# Autodesk Inventor assembly: Tamale Assembly Plate Assembly V3
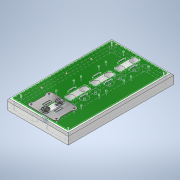
[picture p0: Inventor's stored thumbnail of the model, 180x180]
Saved by Autodesk Inventor 2022 (Build 260153000, 153)
## iProperties
Created: 2022-03-23
Part Number: Tamale Assembly Plate Assembly V3
Document SubType Name: Assembly
Designer: Caleb
Author: Caleb
## Documents named in this file (7)
- C:\Users\Caleb\Desktop\nebraska-silicon-lab\Hardware\ETL\Module Assembly\Tamale Assembly Plate V3\Tamale Assembly Plate Assembly V3.iam
- C:\Users\Caleb\Desktop\nebraska-silicon-lab\Hardware\ETL\Module Assembly\Tamale Assembly Plate V3\Tamale Assembly Plate V3.ipt
- C:\Users\Caleb\Desktop\nebraska-silicon-lab\Hardware\ETL\Module Assembly\Tamale Assembly Plate V3\5427A624_Vacuum Cup.ipt
- C:\Users\Caleb\Desktop\nebraska-silicon-lab\Hardware\ETL\Module Assembly\Tamale Assembly Plate V3\spacer.ipt
- C:\Users\Caleb\Desktop\nebraska-silicon-lab\Hardware\ETL\Module Assembly\Tamale Assembly Plate V3\Assembly Plate PCB.ipt
- C:\Users\Caleb\Desktop\nebraska-silicon-lab\Hardware\ETL\Module Assembly\Tamale Assembly Plate V3\91771A054_Passivated 18-8 Stainless Steel Phillips Flat Head Screw.ipt
- C:\Users\Caleb\Desktop\nebraska-silicon-lab\Hardware\ETL\Module Assembly\Tamale Assembly Plate V3\90910A443_BUTTON HEAD TORX SCREWS.ipt
## Components (13 placed, 6 different names)
1. Tamale Assembly Plate V3:1 — Angle:1, Insert:1, Mate:1, Flush:1, Flush:2, Insert:14
2. 5427A624_Vacuum Cup:1 — Angle:1, Insert:1
3. spacer:1 — Insert:4, Insert:5, Insert:6, Insert:7, Insert:12, Insert:13
4. Assembly Plate PCB:1 — Mate:1, Flush:1, Flush:2, Insert:8, Insert:9, Insert:10, Insert:11, Insert:12, Insert:13
5. 91771A054_Passivated 18-8 Stainless Steel Phillips Flat Head Screw:1 — Insert:4
6. 91771A054_Passivated 18-8 Stainless Steel Phillips Flat Head Screw:2 — Insert:5
7. 91771A054_Passivated 18-8 Stainless Steel Phillips Flat Head Screw:3 — Insert:6
8. 91771A054_Passivated 18-8 Stainless Steel Phillips Flat Head Screw:4 — Insert:7
9. 90910A443_BUTTON HEAD TORX SCREWS:1 — Insert:8
10. 90910A443_BUTTON HEAD TORX SCREWS:2 — Insert:9
11. 90910A443_BUTTON HEAD TORX SCREWS:3 — Insert:10
12. 90910A443_BUTTON HEAD TORX SCREWS:4 — Insert:11
13. 5427A624_Vacuum Cup:2 — Insert:14
## Relationships (16: Insert 12, Flush 2, Angle 1, Mate 1)
- Angle:1 (0 deg): Tamale Assembly Plate V3:1 ↔ 5427A624_Vacuum Cup:1
- Insert:1: Tamale Assembly Plate V3:1 ↔ 5427A624_Vacuum Cup:1
- Mate:1: Tamale Assembly Plate V3:1 ↔ Assembly Plate PCB:1
- Insert:4: spacer:1 ↔ 91771A054_Passivated 18-8 Stainless Steel Phillips Flat Head Screw:1
- Insert:5: spacer:1 ↔ 91771A054_Passivated 18-8 Stainless Steel Phillips Flat Head Screw:2
- Insert:6: spacer:1 ↔ 91771A054_Passivated 18-8 Stainless Steel Phillips Flat Head Screw:3
- Insert:7: spacer:1 ↔ 91771A054_Passivated 18-8 Stainless Steel Phillips Flat Head Screw:4
- Flush:1 (6.35 mm): Tamale Assembly Plate V3:1 ↔ Assembly Plate PCB:1
- Flush:2 (6.35 mm): Tamale Assembly Plate V3:1 ↔ Assembly Plate PCB:1
- Insert:8: Assembly Plate PCB:1 ↔ 90910A443_BUTTON HEAD TORX SCREWS:1
- Insert:9: Assembly Plate PCB:1 ↔ 90910A443_BUTTON HEAD TORX SCREWS:2
- Insert:10: Assembly Plate PCB:1 ↔ 90910A443_BUTTON HEAD TORX SCREWS:3
- Insert:11: Assembly Plate PCB:1 ↔ 90910A443_BUTTON HEAD TORX SCREWS:4
- Insert:12: spacer:1 ↔ Assembly Plate PCB:1
- Insert:13: spacer:1 ↔ Assembly Plate PCB:1
- Insert:14: Tamale Assembly Plate V3:1 ↔ 5427A624_Vacuum Cup:2
